# Autodesk Inventor assembly: DERIVER_INSIDE_CR,REV_ENG
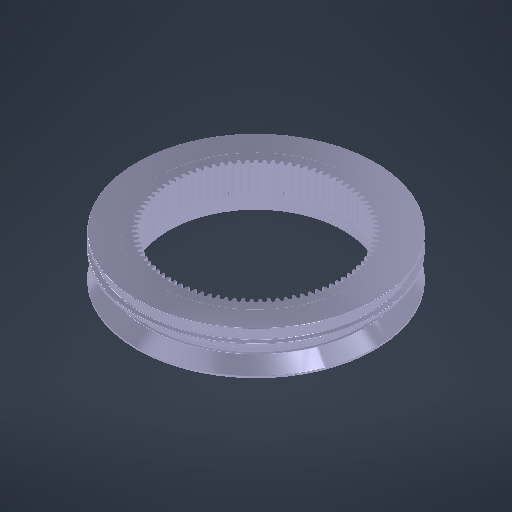
[picture p0: Inventor's stored thumbnail of the model, 512x512]
Saved by Autodesk Inventor 2026.2 (Build 302298010, 298A)
## iProperties
Created: 2026-03-06
Part Number: DERIVER_INSIDE_CR,REV_ENG
Document SubType Name: Assembly
Designer: 4aida
Author: 4aida
## Documents named in this file (3)
- C:\Users\4aida\OneDrive\Documents\GitHub\Design_II_Group6\REV_ENG\DERIVER_INSIDE_CR,REV_ENG.iam
- C:\Users\4aida\OneDrive\Documents\GitHub\Design_II_Group6\REV_ENG\CIRCULAR_SPLINE,REV-ENG.iam
- C:\Users\4aida\OneDrive\Documents\GitHub\Design_II_Group6\REV_ENG\INSIDE_CR_BEARING,REV-ENG.ipt
## Components (2 placed, 2 different names)
1. CIRCULAR_SPLINE,REV-ENG:1 [sub-assembly] — Mate:1, Flush:1
2. INSIDE_CR_BEARING,REV-ENG:1 — Mate:1, Flush:1
## Relationships (2: Mate 1, Flush 1)
- Mate:1: CIRCULAR_SPLINE,REV-ENG:1 ↔ INSIDE_CR_BEARING,REV-ENG:1
- Flush:1: CIRCULAR_SPLINE,REV-ENG:1 ↔ INSIDE_CR_BEARING,REV-ENG:1
